# Autodesk Inventor assembly: BG103_trajan20_21
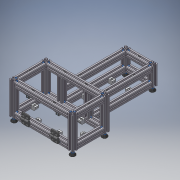
[picture p0: Inventor's stored thumbnail of the model, 180x180]
Saved by Autodesk Inventor 2022.2 (Build 262287000, 287)
## iProperties
Company: HTBLA Kaindorf
RuleStatus: InUse
Created: 2022-08-20
Part Number: BG103_trajan20_21
Project: Zeichenmaschine_v2
Material: Generisch
Description: Gerüst_Step->Bauteil
Document SubType Name: Assembly
Designer: trajan20
AfterDocNew0: iProperties-Editor_aufrufen
Author: jan
Keywords: 2021
## Documents named in this file (7)
- C:\Users\jan\Documents\DrawMachine\DrawMachineConstruction\Projekt\Zeichenmaschine_v2\BG103_trajan20_21_Zeichenmaschine_v2_Gerüst_Step_zu_Bauteil.iam
- C:\Users\jan\Documents\DrawMachine\DrawMachineConstruction\Projekt\Zeichenmaschine_v2\step dateien\gerüst_item_2022-07-24_alu_construct_Projekt_ID-a403a0fdf3734c62922616c2a250de6220_1.ipt
- C:\Users\jan\Documents\DrawMachine\DrawMachineConstruction\Projekt\Zeichenmaschine_v2\step dateien\Magnetschnäpper _093094.ipt
- C:\Users\jan\Documents\DrawMachine\DrawMachineConstruction\Projekt\Zeichenmaschine_v2\step dateien\uniblock_094411m4.ipt
- C:\Users\jan\Documents\DrawMachine\DrawMachineConstruction\Projekt\Zeichenmaschine_v2\step dateien\scharnier_095K2020L00.ipt
- C:\Users\jan\Documents\DrawMachine\DrawMachineConstruction\Projekt\Zeichenmaschine_v2\step dateien\M4_Nutenstein_096214.ipt
- C:\Users\jan\Documents\DrawMachine\DrawMachineConstruction\Projekt\Zeichenmaschine_v2\step dateien\M5_Nutenstein_096215.ipt
## Components (36 placed, 6 different names)
1. gerüst_item_2022-07-24_alu_construct_Projekt_ID-a403a0fdf3734c62922616c2a250de6220_1:1 — Passend:1, Passend:2, Fluchtend:1, Passend:3, Fluchtend:2, Passend:4, Passend:5, Passend:6, Passend:7, Passend:8, Passend:9, Passend:10, Passend:11, Passend:12, Passend:13, Passend:14, Passend:15, Passend:16, Passend:17, Passend:18, Passend:19, Passend:20, Passend:21, Passend:22, Passend:23, Passend:24, Passend:25, Passend:26, Passend:27, Passend:28, Passend:29, Passend:30, Passend:31, Passend:32, Passend:33, Passend:34, Passend:35, Passend:36, Passend:39, Passend:40, Passend:41, Passend:42, Passend:43, Passend:44, Passend:45, Passend:47, Passend:48, Passend:49, Passend:50, Passend:51, Passend:52, Passend:53, Passend:54, Passend:55, Winkel:1, Winkel:2, Passend:57, Winkel:3, Winkel:4, Passend:61, Passend:62, Passend:63, Passend:64, Passend:65, Winkel:5, Passend:66, Winkel:6, Passend:67, Winkel:7, Winkel:8, Passend:70, Passend:71, Winkel:9, Winkel:10, Passend:75, Winkel:11, Passend:76, Passend:78, Passend:79, Passend:80, Passend:81, Passend:82, Winkel:12, Passend:83, Winkel:13, Passend:84, Passend:85, Passend:86, Passend:87, Passend:88, Passend:89, Passend:90, Passend:91, Passend:92, Passend:93, Passend:94, Passend:95, Winkel:14, Winkel:15, Winkel:16, Winkel:17, Passend:96, Passend:97, Winkel:18, Passend:98, Passend:99, Passend:100, Passend:101, Winkel:19, Passend:105
2. Magnetschnäpper _093094:1 — Passend:1, Passend:2, Fluchtend:1, Passend:56, Passend:58
3. Magnetschnäpper _093094:2 — Passend:3, Fluchtend:2, Passend:4, Passend:72, Passend:73
4. uniblock_094411m4:1 — Passend:5, Passend:6, Passend:61
5. uniblock_094411m4:2 — Passend:7, Passend:10, Passend:32
6. uniblock_094411m4:3 — Passend:8, Passend:9, Passend:33
7. uniblock_094411m4:4 — Passend:11, Passend:12, Passend:31
8. uniblock_094411m4:5 — Passend:13, Passend:14, Passend:65
9. uniblock_094411m4:6 — Passend:15, Passend:16, Passend:64
10. uniblock_094411m4:7 — Passend:17, Passend:20, Passend:105
11. uniblock_094411m4:8 — Passend:19, Passend:22, Passend:62
12. uniblock_094411m4:9 — Passend:18, Passend:21, Passend:63
13. uniblock_094411m4:10 — Passend:23, Passend:24, Passend:34
14. uniblock_094411m4:11 — Passend:25, Passend:26, Passend:30
15. uniblock_094411m4:12 — Passend:27, Passend:28, Passend:29
16. scharnier_095K2020L00:1 — Passend:35, Passend:41, Passend:42, Passend:43, Passend:59, Passend:60
17. scharnier_095K2020L00:2 — Passend:36, Passend:39, Passend:40, Passend:44, Passend:68, Passend:69
18. M4_Nutenstein_096214:1 — Passend:45, Winkel:1, Passend:56
19. M4_Nutenstein_096214:3 — Passend:47, Winkel:3, Passend:59
20. M4_Nutenstein_096214:4 — Passend:48, Winkel:4, Passend:60
21. M4_Nutenstein_096214:5 — Passend:49, Winkel:7, Passend:68
22. M4_Nutenstein_096214:6 — Passend:50, Winkel:8, Passend:69
23. M5_Nutenstein_096215:1 — Passend:51, Passend:54, Winkel:6, Passend:67
24. M5_Nutenstein_096215:2 — Passend:52, Passend:53, Winkel:5, Passend:66
25. M5_Nutenstein_096215:3 — Passend:55, Passend:75, Winkel:11, Passend:76
26. M4_Nutenstein_096214:7 — Winkel:2, Passend:57, Passend:58
27. M4_Nutenstein_096214:8 — Passend:70, Winkel:9, Passend:73
28. M4_Nutenstein_096214:9 — Passend:71, Winkel:10, Passend:72
29. M5_Nutenstein_096215:4 — Passend:78, Passend:79, Passend:83, Winkel:13
30. M5_Nutenstein_096215:5 — Passend:80, Passend:81, Passend:82, Winkel:12
31. M5_Nutenstein_096215:6 — Passend:87, Passend:93, Passend:95, Winkel:17
32. M5_Nutenstein_096215:7 — Passend:86, Passend:90, Passend:91, Winkel:14
33. M5_Nutenstein_096215:8 — Passend:85, Passend:92, Passend:94, Winkel:16
34. M5_Nutenstein_096215:9 — Passend:84, Passend:88, Passend:89, Winkel:15
35. M5_Nutenstein_096215:10 — Passend:99, Passend:100, Passend:101, Winkel:19
36. M5_Nutenstein_096215:11 — Passend:96, Passend:97, Winkel:18, Passend:98
## Relationships (118: Mate 97, Angle 19, Flush 2)
- Passend:1 [Mate]: gerüst_item_2022-07-24_alu_construct_Projekt_ID-a403a0fdf3734c62922616c2a250de6220_1:1 ↔ Magnetschnäpper _093094:1
- Passend:2 [Mate] (30 mm): gerüst_item_2022-07-24_alu_construct_Projekt_ID-a403a0fdf3734c62922616c2a250de6220_1:1 ↔ Magnetschnäpper _093094:1
- Fluchtend:1 [Flush] (-1 mm): gerüst_item_2022-07-24_alu_construct_Projekt_ID-a403a0fdf3734c62922616c2a250de6220_1:1 ↔ Magnetschnäpper _093094:1
- Passend:3 [Mate]: gerüst_item_2022-07-24_alu_construct_Projekt_ID-a403a0fdf3734c62922616c2a250de6220_1:1 ↔ Magnetschnäpper _093094:2
- Fluchtend:2 [Flush] (-1 mm): gerüst_item_2022-07-24_alu_construct_Projekt_ID-a403a0fdf3734c62922616c2a250de6220_1:1 ↔ Magnetschnäpper _093094:2
- Passend:4 [Mate] (30 mm): gerüst_item_2022-07-24_alu_construct_Projekt_ID-a403a0fdf3734c62922616c2a250de6220_1:1 ↔ Magnetschnäpper _093094:2
- Passend:5 [Mate]: gerüst_item_2022-07-24_alu_construct_Projekt_ID-a403a0fdf3734c62922616c2a250de6220_1:1 ↔ uniblock_094411m4:1
- Passend:6 [Mate]: gerüst_item_2022-07-24_alu_construct_Projekt_ID-a403a0fdf3734c62922616c2a250de6220_1:1 ↔ uniblock_094411m4:1
- Passend:7 [Mate]: gerüst_item_2022-07-24_alu_construct_Projekt_ID-a403a0fdf3734c62922616c2a250de6220_1:1 ↔ uniblock_094411m4:2
- Passend:8 [Mate]: gerüst_item_2022-07-24_alu_construct_Projekt_ID-a403a0fdf3734c62922616c2a250de6220_1:1 ↔ uniblock_094411m4:3
- Passend:9 [Mate]: gerüst_item_2022-07-24_alu_construct_Projekt_ID-a403a0fdf3734c62922616c2a250de6220_1:1 ↔ uniblock_094411m4:3
- Passend:10 [Mate]: gerüst_item_2022-07-24_alu_construct_Projekt_ID-a403a0fdf3734c62922616c2a250de6220_1:1 ↔ uniblock_094411m4:2
- Passend:11 [Mate]: gerüst_item_2022-07-24_alu_construct_Projekt_ID-a403a0fdf3734c62922616c2a250de6220_1:1 ↔ uniblock_094411m4:4
- Passend:12 [Mate]: gerüst_item_2022-07-24_alu_construct_Projekt_ID-a403a0fdf3734c62922616c2a250de6220_1:1 ↔ uniblock_094411m4:4
- Passend:13 [Mate]: gerüst_item_2022-07-24_alu_construct_Projekt_ID-a403a0fdf3734c62922616c2a250de6220_1:1 ↔ uniblock_094411m4:5
- Passend:14 [Mate]: gerüst_item_2022-07-24_alu_construct_Projekt_ID-a403a0fdf3734c62922616c2a250de6220_1:1 ↔ uniblock_094411m4:5
- Passend:15 [Mate]: gerüst_item_2022-07-24_alu_construct_Projekt_ID-a403a0fdf3734c62922616c2a250de6220_1:1 ↔ uniblock_094411m4:6
- Passend:16 [Mate]: gerüst_item_2022-07-24_alu_construct_Projekt_ID-a403a0fdf3734c62922616c2a250de6220_1:1 ↔ uniblock_094411m4:6
- Passend:17 [Mate]: gerüst_item_2022-07-24_alu_construct_Projekt_ID-a403a0fdf3734c62922616c2a250de6220_1:1 ↔ uniblock_094411m4:7
- Passend:18 [Mate]: gerüst_item_2022-07-24_alu_construct_Projekt_ID-a403a0fdf3734c62922616c2a250de6220_1:1 ↔ uniblock_094411m4:9
- Passend:19 [Mate]: gerüst_item_2022-07-24_alu_construct_Projekt_ID-a403a0fdf3734c62922616c2a250de6220_1:1 ↔ uniblock_094411m4:8
- Passend:20 [Mate]: gerüst_item_2022-07-24_alu_construct_Projekt_ID-a403a0fdf3734c62922616c2a250de6220_1:1 ↔ uniblock_094411m4:7
- Passend:21 [Mate]: gerüst_item_2022-07-24_alu_construct_Projekt_ID-a403a0fdf3734c62922616c2a250de6220_1:1 ↔ uniblock_094411m4:9
- Passend:22 [Mate]: gerüst_item_2022-07-24_alu_construct_Projekt_ID-a403a0fdf3734c62922616c2a250de6220_1:1 ↔ uniblock_094411m4:8
- Passend:23 [Mate]: gerüst_item_2022-07-24_alu_construct_Projekt_ID-a403a0fdf3734c62922616c2a250de6220_1:1 ↔ uniblock_094411m4:10
- Passend:24 [Mate]: gerüst_item_2022-07-24_alu_construct_Projekt_ID-a403a0fdf3734c62922616c2a250de6220_1:1 ↔ uniblock_094411m4:10
- Passend:25 [Mate]: gerüst_item_2022-07-24_alu_construct_Projekt_ID-a403a0fdf3734c62922616c2a250de6220_1:1 ↔ uniblock_094411m4:11
- Passend:26 [Mate]: gerüst_item_2022-07-24_alu_construct_Projekt_ID-a403a0fdf3734c62922616c2a250de6220_1:1 ↔ uniblock_094411m4:11
- Passend:27 [Mate]: gerüst_item_2022-07-24_alu_construct_Projekt_ID-a403a0fdf3734c62922616c2a250de6220_1:1 ↔ uniblock_094411m4:12
- Passend:28 [Mate]: gerüst_item_2022-07-24_alu_construct_Projekt_ID-a403a0fdf3734c62922616c2a250de6220_1:1 ↔ uniblock_094411m4:12
- Passend:29 [Mate] (60 mm): gerüst_item_2022-07-24_alu_construct_Projekt_ID-a403a0fdf3734c62922616c2a250de6220_1:1 ↔ uniblock_094411m4:12
- Passend:30 [Mate] (60 mm): gerüst_item_2022-07-24_alu_construct_Projekt_ID-a403a0fdf3734c62922616c2a250de6220_1:1 ↔ uniblock_094411m4:11
- Passend:31 [Mate] (40 mm): gerüst_item_2022-07-24_alu_construct_Projekt_ID-a403a0fdf3734c62922616c2a250de6220_1:1 ↔ uniblock_094411m4:4
- Passend:32 [Mate] (60 mm): gerüst_item_2022-07-24_alu_construct_Projekt_ID-a403a0fdf3734c62922616c2a250de6220_1:1 ↔ uniblock_094411m4:2
- Passend:33 [Mate] (60 mm): gerüst_item_2022-07-24_alu_construct_Projekt_ID-a403a0fdf3734c62922616c2a250de6220_1:1 ↔ uniblock_094411m4:3
- Passend:34 [Mate] (50 mm): gerüst_item_2022-07-24_alu_construct_Projekt_ID-a403a0fdf3734c62922616c2a250de6220_1:1 ↔ uniblock_094411m4:10
- Passend:35 [Mate]: gerüst_item_2022-07-24_alu_construct_Projekt_ID-a403a0fdf3734c62922616c2a250de6220_1:1 ↔ scharnier_095K2020L00:1
- Passend:36 [Mate] (2.5 mm): gerüst_item_2022-07-24_alu_construct_Projekt_ID-a403a0fdf3734c62922616c2a250de6220_1:1 ↔ scharnier_095K2020L00:2
- Passend:39 [Mate]: gerüst_item_2022-07-24_alu_construct_Projekt_ID-a403a0fdf3734c62922616c2a250de6220_1:1 ↔ scharnier_095K2020L00:2
- Passend:40 [Mate] (2.5 mm): gerüst_item_2022-07-24_alu_construct_Projekt_ID-a403a0fdf3734c62922616c2a250de6220_1:1 ↔ scharnier_095K2020L00:2
- Passend:41 [Mate] (2.5 mm): gerüst_item_2022-07-24_alu_construct_Projekt_ID-a403a0fdf3734c62922616c2a250de6220_1:1 ↔ scharnier_095K2020L00:1
- Passend:42 [Mate] (2.5 mm): gerüst_item_2022-07-24_alu_construct_Projekt_ID-a403a0fdf3734c62922616c2a250de6220_1:1 ↔ scharnier_095K2020L00:1
- Passend:43 [Mate] (30 mm): gerüst_item_2022-07-24_alu_construct_Projekt_ID-a403a0fdf3734c62922616c2a250de6220_1:1 ↔ scharnier_095K2020L00:1
- Passend:44 [Mate] (30 mm): gerüst_item_2022-07-24_alu_construct_Projekt_ID-a403a0fdf3734c62922616c2a250de6220_1:1 ↔ scharnier_095K2020L00:2
- Passend:45 [Mate]: gerüst_item_2022-07-24_alu_construct_Projekt_ID-a403a0fdf3734c62922616c2a250de6220_1:1 ↔ M4_Nutenstein_096214:1
- Passend:47 [Mate]: gerüst_item_2022-07-24_alu_construct_Projekt_ID-a403a0fdf3734c62922616c2a250de6220_1:1 ↔ M4_Nutenstein_096214:3
- Passend:48 [Mate]: gerüst_item_2022-07-24_alu_construct_Projekt_ID-a403a0fdf3734c62922616c2a250de6220_1:1 ↔ M4_Nutenstein_096214:4
- Passend:49 [Mate]: gerüst_item_2022-07-24_alu_construct_Projekt_ID-a403a0fdf3734c62922616c2a250de6220_1:1 ↔ M4_Nutenstein_096214:5
- Passend:50 [Mate]: gerüst_item_2022-07-24_alu_construct_Projekt_ID-a403a0fdf3734c62922616c2a250de6220_1:1 ↔ M4_Nutenstein_096214:6
- Passend:51 [Mate]: gerüst_item_2022-07-24_alu_construct_Projekt_ID-a403a0fdf3734c62922616c2a250de6220_1:1 ↔ M5_Nutenstein_096215:1
- Passend:52 [Mate]: gerüst_item_2022-07-24_alu_construct_Projekt_ID-a403a0fdf3734c62922616c2a250de6220_1:1 ↔ M5_Nutenstein_096215:2
- Passend:53 [Mate] (2.5 mm): gerüst_item_2022-07-24_alu_construct_Projekt_ID-a403a0fdf3734c62922616c2a250de6220_1:1 ↔ M5_Nutenstein_096215:2
- Passend:54 [Mate] (2.5 mm): gerüst_item_2022-07-24_alu_construct_Projekt_ID-a403a0fdf3734c62922616c2a250de6220_1:1 ↔ M5_Nutenstein_096215:1
- Passend:55 [Mate]: gerüst_item_2022-07-24_alu_construct_Projekt_ID-a403a0fdf3734c62922616c2a250de6220_1:1 ↔ M5_Nutenstein_096215:3
- Winkel:1 [Angle] (180 deg): gerüst_item_2022-07-24_alu_construct_Projekt_ID-a403a0fdf3734c62922616c2a250de6220_1:1 ↔ M4_Nutenstein_096214:1
- Passend:56 [Mate]: Magnetschnäpper _093094:1 ↔ M4_Nutenstein_096214:1
- Winkel:2 [Angle] (0 deg): gerüst_item_2022-07-24_alu_construct_Projekt_ID-a403a0fdf3734c62922616c2a250de6220_1:1 ↔ M4_Nutenstein_096214:7
- Passend:57 [Mate]: gerüst_item_2022-07-24_alu_construct_Projekt_ID-a403a0fdf3734c62922616c2a250de6220_1:1 ↔ M4_Nutenstein_096214:7
- Passend:58 [Mate]: Magnetschnäpper _093094:1 ↔ M4_Nutenstein_096214:7
- Winkel:3 [Angle] (0 deg): gerüst_item_2022-07-24_alu_construct_Projekt_ID-a403a0fdf3734c62922616c2a250de6220_1:1 ↔ M4_Nutenstein_096214:3
- Passend:59 [Mate]: scharnier_095K2020L00:1 ↔ M4_Nutenstein_096214:3
- Winkel:4 [Angle] (0 deg): gerüst_item_2022-07-24_alu_construct_Projekt_ID-a403a0fdf3734c62922616c2a250de6220_1:1 ↔ M4_Nutenstein_096214:4
- Passend:60 [Mate]: scharnier_095K2020L00:1 ↔ M4_Nutenstein_096214:4
- Passend:61 [Mate] (50 mm): gerüst_item_2022-07-24_alu_construct_Projekt_ID-a403a0fdf3734c62922616c2a250de6220_1:1 ↔ uniblock_094411m4:1
- Passend:62 [Mate] (60 mm): gerüst_item_2022-07-24_alu_construct_Projekt_ID-a403a0fdf3734c62922616c2a250de6220_1:1 ↔ uniblock_094411m4:8
- Passend:63 [Mate] (60 mm): gerüst_item_2022-07-24_alu_construct_Projekt_ID-a403a0fdf3734c62922616c2a250de6220_1:1 ↔ uniblock_094411m4:9
- Passend:64 [Mate] (60 mm): gerüst_item_2022-07-24_alu_construct_Projekt_ID-a403a0fdf3734c62922616c2a250de6220_1:1 ↔ uniblock_094411m4:6
- Passend:65 [Mate] (60 mm): gerüst_item_2022-07-24_alu_construct_Projekt_ID-a403a0fdf3734c62922616c2a250de6220_1:1 ↔ uniblock_094411m4:5
- Winkel:5 [Angle] (0 deg): gerüst_item_2022-07-24_alu_construct_Projekt_ID-a403a0fdf3734c62922616c2a250de6220_1:1 ↔ M5_Nutenstein_096215:2
- Passend:66 [Mate] (60 mm): gerüst_item_2022-07-24_alu_construct_Projekt_ID-a403a0fdf3734c62922616c2a250de6220_1:1 ↔ M5_Nutenstein_096215:2
- Winkel:6 [Angle] (0 deg): gerüst_item_2022-07-24_alu_construct_Projekt_ID-a403a0fdf3734c62922616c2a250de6220_1:1 ↔ M5_Nutenstein_096215:1
- Passend:67 [Mate] (60 mm): gerüst_item_2022-07-24_alu_construct_Projekt_ID-a403a0fdf3734c62922616c2a250de6220_1:1 ↔ M5_Nutenstein_096215:1
- Winkel:7 [Angle] (180 deg): gerüst_item_2022-07-24_alu_construct_Projekt_ID-a403a0fdf3734c62922616c2a250de6220_1:1 ↔ M4_Nutenstein_096214:5
- Passend:68 [Mate]: scharnier_095K2020L00:2 ↔ M4_Nutenstein_096214:5
- Winkel:8 [Angle] (180 deg): gerüst_item_2022-07-24_alu_construct_Projekt_ID-a403a0fdf3734c62922616c2a250de6220_1:1 ↔ M4_Nutenstein_096214:6
- Passend:69 [Mate]: scharnier_095K2020L00:2 ↔ M4_Nutenstein_096214:6
- Passend:70 [Mate]: gerüst_item_2022-07-24_alu_construct_Projekt_ID-a403a0fdf3734c62922616c2a250de6220_1:1 ↔ M4_Nutenstein_096214:8
- Passend:71 [Mate]: gerüst_item_2022-07-24_alu_construct_Projekt_ID-a403a0fdf3734c62922616c2a250de6220_1:1 ↔ M4_Nutenstein_096214:9
- Winkel:9 [Angle] (0 deg): gerüst_item_2022-07-24_alu_construct_Projekt_ID-a403a0fdf3734c62922616c2a250de6220_1:1 ↔ M4_Nutenstein_096214:8
- Winkel:10 [Angle] (180 deg): gerüst_item_2022-07-24_alu_construct_Projekt_ID-a403a0fdf3734c62922616c2a250de6220_1:1 ↔ M4_Nutenstein_096214:9
- Passend:72 [Mate]: Magnetschnäpper _093094:2 ↔ M4_Nutenstein_096214:9
- Passend:73 [Mate]: Magnetschnäpper _093094:2 ↔ M4_Nutenstein_096214:8
- Passend:75 [Mate] (60 mm): gerüst_item_2022-07-24_alu_construct_Projekt_ID-a403a0fdf3734c62922616c2a250de6220_1:1 ↔ M5_Nutenstein_096215:3
- Winkel:11 [Angle] (180 deg): gerüst_item_2022-07-24_alu_construct_Projekt_ID-a403a0fdf3734c62922616c2a250de6220_1:1 ↔ M5_Nutenstein_096215:3
- Passend:76 [Mate] (2.5 mm): gerüst_item_2022-07-24_alu_construct_Projekt_ID-a403a0fdf3734c62922616c2a250de6220_1:1 ↔ M5_Nutenstein_096215:3
- Passend:78 [Mate] (2.5 mm): gerüst_item_2022-07-24_alu_construct_Projekt_ID-a403a0fdf3734c62922616c2a250de6220_1:1 ↔ M5_Nutenstein_096215:4
- Passend:79 [Mate] (60 mm): gerüst_item_2022-07-24_alu_construct_Projekt_ID-a403a0fdf3734c62922616c2a250de6220_1:1 ↔ M5_Nutenstein_096215:4
- Passend:80 [Mate] (40 mm): gerüst_item_2022-07-24_alu_construct_Projekt_ID-a403a0fdf3734c62922616c2a250de6220_1:1 ↔ M5_Nutenstein_096215:5
- Passend:81 [Mate]: gerüst_item_2022-07-24_alu_construct_Projekt_ID-a403a0fdf3734c62922616c2a250de6220_1:1 ↔ M5_Nutenstein_096215:5
- Passend:82 [Mate] (2.5 mm): gerüst_item_2022-07-24_alu_construct_Projekt_ID-a403a0fdf3734c62922616c2a250de6220_1:1 ↔ M5_Nutenstein_096215:5
- Winkel:12 [Angle] (180 deg): gerüst_item_2022-07-24_alu_construct_Projekt_ID-a403a0fdf3734c62922616c2a250de6220_1:1 ↔ M5_Nutenstein_096215:5
- Passend:83 [Mate]: gerüst_item_2022-07-24_alu_construct_Projekt_ID-a403a0fdf3734c62922616c2a250de6220_1:1 ↔ M5_Nutenstein_096215:4
- Winkel:13 [Angle] (180 deg): gerüst_item_2022-07-24_alu_construct_Projekt_ID-a403a0fdf3734c62922616c2a250de6220_1:1 ↔ M5_Nutenstein_096215:4
- Passend:84 [Mate]: gerüst_item_2022-07-24_alu_construct_Projekt_ID-a403a0fdf3734c62922616c2a250de6220_1:1 ↔ M5_Nutenstein_096215:9
- Passend:85 [Mate]: gerüst_item_2022-07-24_alu_construct_Projekt_ID-a403a0fdf3734c62922616c2a250de6220_1:1 ↔ M5_Nutenstein_096215:8
- Passend:86 [Mate]: gerüst_item_2022-07-24_alu_construct_Projekt_ID-a403a0fdf3734c62922616c2a250de6220_1:1 ↔ M5_Nutenstein_096215:7
- Passend:87 [Mate]: gerüst_item_2022-07-24_alu_construct_Projekt_ID-a403a0fdf3734c62922616c2a250de6220_1:1 ↔ M5_Nutenstein_096215:6
- Passend:88 [Mate] (60 mm): gerüst_item_2022-07-24_alu_construct_Projekt_ID-a403a0fdf3734c62922616c2a250de6220_1:1 ↔ M5_Nutenstein_096215:9
- Passend:89 [Mate] (2.5 mm): gerüst_item_2022-07-24_alu_construct_Projekt_ID-a403a0fdf3734c62922616c2a250de6220_1:1 ↔ M5_Nutenstein_096215:9
- Passend:90 [Mate] (2.5 mm): gerüst_item_2022-07-24_alu_construct_Projekt_ID-a403a0fdf3734c62922616c2a250de6220_1:1 ↔ M5_Nutenstein_096215:7
- Passend:91 [Mate] (60 mm): gerüst_item_2022-07-24_alu_construct_Projekt_ID-a403a0fdf3734c62922616c2a250de6220_1:1 ↔ M5_Nutenstein_096215:7
- Passend:92 [Mate] (60 mm): gerüst_item_2022-07-24_alu_construct_Projekt_ID-a403a0fdf3734c62922616c2a250de6220_1:1 ↔ M5_Nutenstein_096215:8
- Passend:93 [Mate] (60 mm): gerüst_item_2022-07-24_alu_construct_Projekt_ID-a403a0fdf3734c62922616c2a250de6220_1:1 ↔ M5_Nutenstein_096215:6
- Passend:94 [Mate] (2.5 mm): gerüst_item_2022-07-24_alu_construct_Projekt_ID-a403a0fdf3734c62922616c2a250de6220_1:1 ↔ M5_Nutenstein_096215:8
- Passend:95 [Mate] (2.5 mm): gerüst_item_2022-07-24_alu_construct_Projekt_ID-a403a0fdf3734c62922616c2a250de6220_1:1 ↔ M5_Nutenstein_096215:6
- Winkel:14 [Angle] (180 deg): gerüst_item_2022-07-24_alu_construct_Projekt_ID-a403a0fdf3734c62922616c2a250de6220_1:1 ↔ M5_Nutenstein_096215:7
- Winkel:15 [Angle] (0 deg): gerüst_item_2022-07-24_alu_construct_Projekt_ID-a403a0fdf3734c62922616c2a250de6220_1:1 ↔ M5_Nutenstein_096215:9
- Winkel:16 [Angle] (0 deg): gerüst_item_2022-07-24_alu_construct_Projekt_ID-a403a0fdf3734c62922616c2a250de6220_1:1 ↔ M5_Nutenstein_096215:8
- Winkel:17 [Angle] (0 deg): gerüst_item_2022-07-24_alu_construct_Projekt_ID-a403a0fdf3734c62922616c2a250de6220_1:1 ↔ M5_Nutenstein_096215:6
- Passend:96 [Mate]: gerüst_item_2022-07-24_alu_construct_Projekt_ID-a403a0fdf3734c62922616c2a250de6220_1:1 ↔ M5_Nutenstein_096215:11
- Passend:97 [Mate] (2.5 mm): gerüst_item_2022-07-24_alu_construct_Projekt_ID-a403a0fdf3734c62922616c2a250de6220_1:1 ↔ M5_Nutenstein_096215:11
- Winkel:18 [Angle] (0 deg): gerüst_item_2022-07-24_alu_construct_Projekt_ID-a403a0fdf3734c62922616c2a250de6220_1:1 ↔ M5_Nutenstein_096215:11
- Passend:98 [Mate] (50 mm): gerüst_item_2022-07-24_alu_construct_Projekt_ID-a403a0fdf3734c62922616c2a250de6220_1:1 ↔ M5_Nutenstein_096215:11
- Passend:99 [Mate] (50 mm): gerüst_item_2022-07-24_alu_construct_Projekt_ID-a403a0fdf3734c62922616c2a250de6220_1:1 ↔ M5_Nutenstein_096215:10
- Passend:100 [Mate]: gerüst_item_2022-07-24_alu_construct_Projekt_ID-a403a0fdf3734c62922616c2a250de6220_1:1 ↔ M5_Nutenstein_096215:10
- Passend:101 [Mate] (2.5 mm): gerüst_item_2022-07-24_alu_construct_Projekt_ID-a403a0fdf3734c62922616c2a250de6220_1:1 ↔ M5_Nutenstein_096215:10
- Winkel:19 [Angle] (0 deg): gerüst_item_2022-07-24_alu_construct_Projekt_ID-a403a0fdf3734c62922616c2a250de6220_1:1 ↔ M5_Nutenstein_096215:10
- Passend:105 [Mate] (40 mm): gerüst_item_2022-07-24_alu_construct_Projekt_ID-a403a0fdf3734c62922616c2a250de6220_1:1 ↔ uniblock_094411m4:7
